# Autodesk Inventor assembly: Force_plate
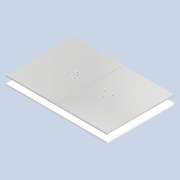
[picture p0: Inventor's stored thumbnail of the model, 180x180]
Saved by Autodesk Inventor 2022 (Build 260153000, 153)
## iProperties
Created: 2023-06-20
Part Number: Force_plate
Document SubType Name: Assembly
Designer: 81805
Author: 81805
## Documents named in this file (5)
- D:\GitHub\inventor\ForcePlate\Force_plate.iam
- D:\GitHub\inventor\ForcePlate\FFS080YS102U6.ipt
- D:\GitHub\inventor\ForcePlate\Board.ipt
- D:\GitHub\inventor\ForcePlate\Bottom_board.ipt
- D:\GitHub\inventor\ForcePlate\M6-12.ipt
## Components (11 placed, 4 different names)
1. FFS080YS102U6:1 — メイト:5, 角度:1, 角度:2, メイト:7, 挿入:7
2. FFS080YS102U6:2 — メイト:6, 角度:3, 角度:4, メイト:7, 挿入:8
3. Board:1 — フラッシュ:2, フラッシュ:3, 挿入:7
4. Board:2 — フラッシュ:1, 挿入:8
5. Bottom_board:1 — メイト:5, メイト:6, フラッシュ:1, フラッシュ:2, フラッシュ:3
6. M6-12:1
7. M6-12:2
8. M6-12:3
9. M6-12:4
10. M6-12:5
11. M6-12:6
## Relationships (18: Insert 8, Angle 4, Mate 3, Flush 3)
- メイト:5 [Mate]: FFS080YS102U6:1 ↔ Bottom_board:1
- メイト:6 [Mate]: FFS080YS102U6:2 ↔ Bottom_board:1
- フラッシュ:1 [Flush]: Board:2 ↔ Bottom_board:1
- フラッシュ:2 [Flush]: Board:1 ↔ Bottom_board:1
- 角度:1 [Angle] (0 deg): FFS080YS102U6:1
- 角度:2 [Angle] (180 deg): FFS080YS102U6:1
- 角度:3 [Angle] (0 deg): FFS080YS102U6:2
- 角度:4 [Angle] (180 deg): FFS080YS102U6:2
- メイト:7 [Mate] (20 mm): FFS080YS102U6:1 ↔ FFS080YS102U6:2
- フラッシュ:3 [Flush]: Board:1 ↔ Bottom_board:1
- [Insert]: Board:2 ↔ M6-12:6
- [Insert]: Board:2 ↔ M6-12:5
- [Insert]: Board:1 ↔ M6-12:4
- [Insert]: Board:1 ↔ M6-12:2
- [Insert]: Board:1 ↔ M6-12:1
- [Insert]: Board:2 ↔ M6-12:3
- 挿入:7 [Insert]: FFS080YS102U6:1 ↔ Board:1
- 挿入:8 [Insert]: FFS080YS102U6:2 ↔ Board:2
